# Autodesk Inventor assembly: TreadAssembly_MIR
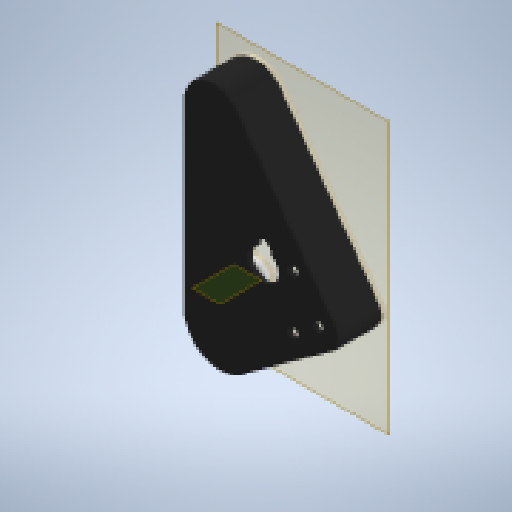
[picture p0: Inventor's stored thumbnail of the model, 512x512]
Saved by Autodesk Inventor 2025.2 (Build 292293000, 293)
## iProperties
Created: 2025-01-27
Part Number: TreadAssembly_MIR
Document SubType Name: Assembly
Designer: andre
Author: andre
## Documents named in this file (3)
- C:\Users\andre\Documents\GitHub\Handshake\Hardware\Proto2-WallE\TreadAssembly_MIR.iam
- C:\Users\andre\Documents\GitHub\Handshake\Hardware\Proto2-WallE\TreadWheeled_MIR.ipt
- C:\Users\andre\Documents\GitHub\Handshake\Hardware\Proto2-WallE\TreadWheeledCover_MIR.ipt
## Components (2 placed, 2 different names)
1. TreadWheeled_MIR:1 — Flush:2, Flush:1
2. TreadWheeledCover_MIR:1 — Flush:2, Flush:1
## Relationships (2: Mate 2)
- Flush:2 [Mate]: TreadWheeled_MIR:1 ↔ TreadWheeledCover_MIR:1
- Flush:1 [Mate]: TreadWheeled_MIR:1 ↔ TreadWheeledCover_MIR:1
